# Autodesk Inventor assembly: supply
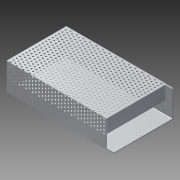
[picture p0: Inventor's stored thumbnail of the model, 180x180]
Saved by Autodesk Inventor 2015 (Build 190159000, 159)
## iProperties
Created: 2015-01-31
Part Number: supply
Document SubType Name: Assembly
Designer: Joseph
Author: Joseph
## Documents named in this file (3)
- Z:\CloudStation\3d models\Kossel\supply.iam
- Z:\CloudStation\3d models\Kossel\supply base.ipt
- Z:\CloudStation\3d models\Kossel\supply shield.ipt
## Components (2 placed, 2 different names)
1. supply base:1 — Flush:1, Flush:2, Flush:3
2. supply shield:1 — Flush:1, Flush:2, Flush:3
## Relationships (3: Flush 3)
- Flush:1: supply base:1 ↔ supply shield:1
- Flush:2: supply base:1 ↔ supply shield:1
- Flush:3: supply base:1 ↔ supply shield:1
